# Autodesk Inventor assembly: Zebro_lotka_normal
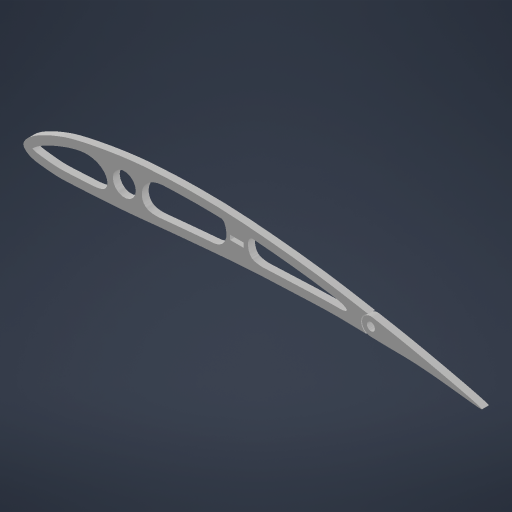
[picture p0: Inventor's stored thumbnail of the model, 512x512]
Saved by Autodesk Inventor 2023 (Build 270158000, 158)
## iProperties
Created: 2022-12-09
Part Number: Zebro_lotka_normal
Document SubType Name: Assembly
Designer: szykr
Author: szykr
## Documents named in this file (3)
- D:\Folder Instalacyjny\GitHub Pliki\Solaris\model\Zebro_lotka_normal.iam
- D:\Folder Instalacyjny\GitHub Pliki\Solaris\model\Żebro z lotką.ipt
- D:\Folder Instalacyjny\GitHub Pliki\Solaris\model\Lotka.ipt
## Components (2 placed, 2 different names)
1. Żebro z lotką:1 — Insert:1
2. Lotka:1 — Insert:1
## Relationships (1: Insert 1)
- Insert:1: Żebro z lotką:1 ↔ Lotka:1
